# Autodesk Inventor assembly: ASY MSC 080 gills
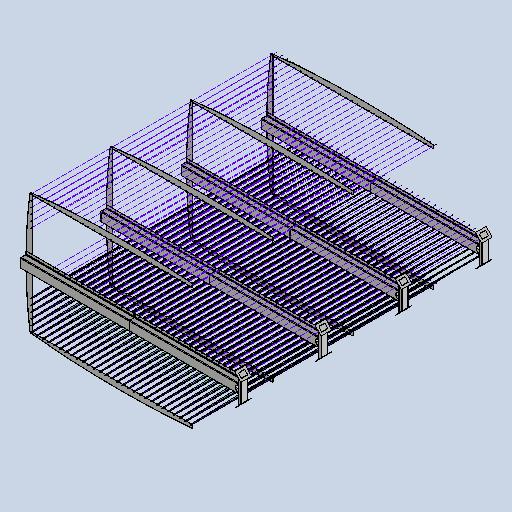
[picture p0: Inventor's stored thumbnail of the model, 512x512]
Saved by Autodesk Inventor 2025 (Build 290162010, 162A)
## iProperties
Created: 2024-08-31
Part Number: ASY MSC 080 gills
Document SubType Name: Assembly
Designer: pokla
Stock Number: ASY МОО 080 Жабры
Author: pokla
## Documents named in this file (20)
- C:\Users\pokla\Documents\Inventor\Отстойник осветлитель\Manturovo_Se-clar-Gleb\ASY MSC Жабры.iam
- C:\Users\pokla\Documents\Inventor\Отстойник осветлитель\Manturovo_Se-clar-Gleb\MSC 802 sheet gills.ipt
- C:\Users\pokla\Documents\Inventor\Отстойник осветлитель\Manturovo_Se-clar-Gleb\MSC 081 pillar gills.ipt
- C:\Users\pokla\Documents\Inventor\Отстойник осветлитель\Manturovo_Se-clar-Gleb\MSC 804 sheet gills.ipt
- C:\Users\pokla\Documents\Inventor\Отстойник осветлитель\Manturovo_Se-clar-Gleb\MSC 803 sheet gills.ipt
- C:\Users\pokla\Documents\Inventor\Отстойник осветлитель\Manturovo_Se-clar-Gleb\MSC 806 sheet gills.ipt
- C:\Users\pokla\Documents\Inventor\Отстойник осветлитель\Manturovo_Se-clar-Gleb\MSC 805 sheet gills.ipt
- C:\Users\pokla\Documents\Inventor\Отстойник осветлитель\Manturovo_Se-clar-Gleb\MSC 808 sheet gills.ipt
- C:\Users\pokla\Documents\Inventor\Отстойник осветлитель\Manturovo_Se-clar-Gleb\MSC 807 sheet gills.ipt
- C:\Users\pokla\Documents\Inventor\Отстойник осветлитель\Manturovo_Se-clar-Gleb\MSC 810 sheet gills.ipt
- C:\Users\pokla\Documents\Inventor\Отстойник осветлитель\Manturovo_Se-clar-Gleb\MSC 809 sheet gills.ipt
- C:\Users\pokla\Documents\Inventor\Отстойник осветлитель\Manturovo_Se-clar-Gleb\MSC 812 sheet gills.ipt
- C:\Users\pokla\Documents\Inventor\Отстойник осветлитель\Manturovo_Se-clar-Gleb\MSC 811 sheet gills.ipt
- C:\Users\pokla\Documents\Inventor\Отстойник осветлитель\Manturovo_Se-clar-Gleb\MSC 084 wall support gills.ipt
- C:\Users\pokla\Documents\Inventor\Отстойник осветлитель\Manturovo_Se-clar-Gleb\MSC 085 bottom support gills.ipt
- C:\Users\pokla\Documents\Inventor\Отстойник осветлитель\Manturovo_Se-clar-Gleb\MSC 082 pillar gills.ipt
- C:\Users\pokla\Documents\Inventor\Отстойник осветлитель\Manturovo_Se-clar-Gleb\MSC 086 string for sheets gills.ipt
- C:\Users\pokla\Documents\Inventor\Отстойник осветлитель\Manturovo_Se-clar-Gleb\MSC 083 top support gills.ipt
- C:\Users\pokla\Documents\Inventor\Отстойник осветлитель\Manturovo_Se-clar-Gleb\MSC 087 bottom plate gills.ipt
- C:\Users\pokla\Documents\Inventor\Отстойник осветлитель\Manturovo_Se-clar-Gleb\MSC 801 sheet gills.ipt
## Components (240 placed, 19 different names)
1. MSC 804 sheet gills:1 — Rigid:39
2. MSC 803 sheet gills:1 — Angle:2, Tangent:8, Tangent:9, Flush:15, Flush:19, Rigid:39
3. MSC 806 sheet gills:1 — Rigid:36
4. MSC 805 sheet gills:1 — Rigid:36, Angle:3, Tangent:10, Tangent:11, Flush:15, Flush:16
5. MSC 808 sheet gills:1 — Rigid:37
6. MSC 807 sheet gills:1 — Rigid:37, Angle:4, Tangent:12, Tangent:13, Flush:16, Flush:17
7. MSC 810 sheet gills:1 — Rigid:38
8. MSC 809 sheet gills:1 — Rigid:38, Angle:5, Tangent:17, Tangent:18, Flush:17, Flush:18
9. MSC 812 sheet gills:1 — Rigid:32
10. MSC 811 sheet gills:1 — Rigid:32, Angle:6, Tangent:19, Tangent:20, Flush:18
11. MSC 084 wall support gills:1 — Rigid:12, Rigid:25, Rigid:30, Tangent:14, Tangent:15
12. MSC 084 wall support gills:2 — Rigid:25, Rigid:26, Mate:17
13. MSC 084 wall support gills:3 — Rigid:26, Rigid:27
14. MSC 084 wall support gills:4 — Rigid:27
15. MSC 085 bottom support gills:1 — Rigid:6, Rigid:7, Flush:12, Mate:12, Flush:14, Mate:15, Mate:16, Flush:9
16. MSC 081 pillar gills:1 — Flush:12, Mate:12, Flush:14, Rotational:1, Rotational:2, Tangent:16
17. MSC 082 pillar gills:1 — Rigid:28, Rigid:29
18. MSC 085 bottom support gills:2
19. MSC 081 pillar gills:2
20. MSC 082 pillar gills:2
21. MSC 085 bottom support gills:3
22. MSC 081 pillar gills:3
23. MSC 082 pillar gills:3
24. MSC 085 bottom support gills:4
25. MSC 081 pillar gills:4
26. MSC 082 pillar gills:4
27. MSC 801 sheet gills:1 — Mate:17, Rigid:33, Angle:2, Angle:3, Angle:4, Angle:5, Angle:6, Tangent:14, Tangent:15, Tangent:16, Flush:19
28. MSC 801 sheet gills:2
29. MSC 801 sheet gills:3
30. MSC 801 sheet gills:4
31. MSC 801 sheet gills:5
32. MSC 801 sheet gills:6
33. MSC 801 sheet gills:7
34. MSC 801 sheet gills:8
35. MSC 801 sheet gills:9
36. MSC 801 sheet gills:10
37. MSC 801 sheet gills:11
38. MSC 801 sheet gills:12
39. MSC 801 sheet gills:13
40. MSC 801 sheet gills:14
41. MSC 801 sheet gills:15
42. MSC 801 sheet gills:16
43. MSC 801 sheet gills:17
44. MSC 801 sheet gills:18
45. MSC 801 sheet gills:19
46. MSC 801 sheet gills:20
47. MSC 801 sheet gills:21
48. MSC 801 sheet gills:22
49. MSC 801 sheet gills:23
50. MSC 801 sheet gills:24
51. MSC 801 sheet gills:25
52. MSC 801 sheet gills:26
53. MSC 801 sheet gills:27
54. MSC 801 sheet gills:28
55. MSC 801 sheet gills:29
56. MSC 802 sheet gills:1 — Rigid:33
57. MSC 802 sheet gills:2
58. MSC 802 sheet gills:3
59. MSC 802 sheet gills:4
60. MSC 802 sheet gills:5
61. MSC 802 sheet gills:6
62. MSC 802 sheet gills:7
63. MSC 802 sheet gills:8
64. MSC 802 sheet gills:9
65. MSC 802 sheet gills:10
66. MSC 802 sheet gills:11
67. MSC 802 sheet gills:12
68. MSC 802 sheet gills:13
69. MSC 802 sheet gills:14
70. MSC 802 sheet gills:15
71. MSC 802 sheet gills:16
72. MSC 802 sheet gills:17
73. MSC 802 sheet gills:18
74. MSC 802 sheet gills:19
75. MSC 802 sheet gills:20
76. MSC 802 sheet gills:21
77. MSC 802 sheet gills:22
78. MSC 802 sheet gills:23
79. MSC 802 sheet gills:24
80. MSC 802 sheet gills:25
81. MSC 802 sheet gills:26
82. MSC 802 sheet gills:27
83. MSC 802 sheet gills:28
84. MSC 802 sheet gills:29
85. MSC 084 wall support gills:5 — Rigid:15, Rigid:31
86. MSC 083 top support gills:1 — Rigid:24, Rigid:29, Rigid:31
87. MSC 083 top support gills:2 — Rigid:28, Rigid:30, Tangent:8, Tangent:9, Tangent:10, Tangent:11, Tangent:12, Tangent:13, Tangent:17, Tangent:18, Tangent:19, Tangent:20, Rigid:40
88. MSC 087 bottom plate gills:1 — Rigid:6
89. MSC 087 bottom plate gills:2 — Rigid:7
90. MSC 084 wall support gills:6
91. MSC 083 top support gills:3
92. MSC 083 top support gills:4
93. MSC 087 bottom plate gills:3
94. MSC 087 bottom plate gills:4
95. MSC 084 wall support gills:7
96. MSC 083 top support gills:5
97. MSC 083 top support gills:6
98. MSC 087 bottom plate gills:5
99. MSC 087 bottom plate gills:6
100. MSC 084 wall support gills:8
101. MSC 083 top support gills:7
102. MSC 083 top support gills:8
103. MSC 087 bottom plate gills:7
104. MSC 087 bottom plate gills:8
105. MSC 086 string for sheets gills:1 — Rigid:12
106. MSC 086 string for sheets gills:2 — Rigid:15
107. MSC 086 string for sheets gills:3
108. MSC 086 string for sheets gills:4
109. MSC 086 string for sheets gills:5
110. MSC 086 string for sheets gills:6
111. MSC 086 string for sheets gills:7
112. MSC 086 string for sheets gills:8
113. MSC 086 string for sheets gills:9
114. MSC 086 string for sheets gills:10
115. MSC 086 string for sheets gills:11
116. MSC 086 string for sheets gills:12
117. MSC 086 string for sheets gills:13
118. MSC 086 string for sheets gills:14
119. MSC 086 string for sheets gills:15
120. MSC 086 string for sheets gills:16
121. MSC 086 string for sheets gills:17
122. MSC 086 string for sheets gills:18
123. MSC 086 string for sheets gills:19
124. MSC 086 string for sheets gills:20
125. MSC 086 string for sheets gills:21
126. MSC 086 string for sheets gills:22
127. MSC 086 string for sheets gills:23
128. MSC 086 string for sheets gills:24
129. MSC 086 string for sheets gills:25
130. MSC 086 string for sheets gills:26
131. MSC 086 string for sheets gills:27
132. MSC 086 string for sheets gills:28
133. MSC 086 string for sheets gills:29
134. MSC 086 string for sheets gills:30
135. MSC 086 string for sheets gills:31
136. MSC 086 string for sheets gills:32
137. MSC 086 string for sheets gills:33
138. MSC 086 string for sheets gills:34
139. MSC 086 string for sheets gills:35
140. MSC 086 string for sheets gills:36
141. MSC 086 string for sheets gills:37
142. MSC 086 string for sheets gills:38
143. MSC 086 string for sheets gills:39
144. MSC 086 string for sheets gills:40
145. MSC 086 string for sheets gills:41
146. MSC 086 string for sheets gills:42
147. MSC 086 string for sheets gills:43
148. MSC 086 string for sheets gills:44
149. MSC 086 string for sheets gills:45
150. MSC 086 string for sheets gills:46
151. MSC 086 string for sheets gills:47
152. MSC 086 string for sheets gills:48
153. MSC 086 string for sheets gills:49
154. MSC 086 string for sheets gills:50
155. MSC 086 string for sheets gills:51
156. MSC 086 string for sheets gills:52
157. MSC 086 string for sheets gills:53
158. MSC 086 string for sheets gills:54
159. MSC 086 string for sheets gills:55
160. MSC 086 string for sheets gills:56
161. MSC 086 string for sheets gills:57 — Rotational:2
162. MSC 086 string for sheets gills:58 — Rotational:1
163. MSC 086 string for sheets gills:59
164. MSC 086 string for sheets gills:60
165. MSC 086 string for sheets gills:61
166. MSC 086 string for sheets gills:62
167. MSC 086 string for sheets gills:63
168. MSC 086 string for sheets gills:64
169. MSC 086 string for sheets gills:65
170. MSC 086 string for sheets gills:66
171. MSC 086 string for sheets gills:67
172. MSC 086 string for sheets gills:68
173. MSC 086 string for sheets gills:69
174. MSC 086 string for sheets gills:70
175. MSC 086 string for sheets gills:71
176. MSC 086 string for sheets gills:72
177. MSC 086 string for sheets gills:73
178. MSC 086 string for sheets gills:74
179. MSC 086 string for sheets gills:75
180. MSC 086 string for sheets gills:76
181. MSC 086 string for sheets gills:77
182. MSC 086 string for sheets gills:78
183. MSC 086 string for sheets gills:79
184. MSC 086 string for sheets gills:80
185. MSC 086 string for sheets gills:81
186. MSC 086 string for sheets gills:82
187. MSC 086 string for sheets gills:83
188. MSC 086 string for sheets gills:84
189. MSC 086 string for sheets gills:85
190. MSC 086 string for sheets gills:86
191. MSC 086 string for sheets gills:87
192. MSC 086 string for sheets gills:88
193. MSC 086 string for sheets gills:89
194. MSC 086 string for sheets gills:90
195. MSC 086 string for sheets gills:91
196. MSC 086 string for sheets gills:92
197. MSC 086 string for sheets gills:93
198. MSC 086 string for sheets gills:94
199. MSC 086 string for sheets gills:95
200. MSC 086 string for sheets gills:96
201. MSC 086 string for sheets gills:97
202. MSC 086 string for sheets gills:98
203. MSC 086 string for sheets gills:99
204. MSC 086 string for sheets gills:100
205. MSC 086 string for sheets gills:101
206. MSC 086 string for sheets gills:102
207. MSC 086 string for sheets gills:103
208. MSC 086 string for sheets gills:104
209. MSC 086 string for sheets gills:105
210. MSC 086 string for sheets gills:106
211. MSC 086 string for sheets gills:107
212. MSC 086 string for sheets gills:108
213. MSC 086 string for sheets gills:109
214. MSC 086 string for sheets gills:110
215. MSC 086 string for sheets gills:111
216. MSC 086 string for sheets gills:112
217. MSC 086 string for sheets gills:113
218. MSC 086 string for sheets gills:114
219. MSC 086 string for sheets gills:115
220. MSC 086 string for sheets gills:116
221. MSC 086 string for sheets gills:117
222. MSC 086 string for sheets gills:118
223. MSC 086 string for sheets gills:119
224. MSC 086 string for sheets gills:120
225. MSC 086 string for sheets gills:121
226. MSC 086 string for sheets gills:122
227. MSC 086 string for sheets gills:123
228. MSC 086 string for sheets gills:124
229. MSC 086 string for sheets gills:125 — Rigid:40
230. MSC 086 string for sheets gills:126
231. MSC 086 string for sheets gills:127
232. MSC 086 string for sheets gills:128
233. MSC 086 string for sheets gills:129
234. MSC 086 string for sheets gills:130
235. MSC 086 string for sheets gills:131 — Rigid:24
236. MSC 086 string for sheets gills:132
237. MSC 086 string for sheets gills:133
238. MSC 086 string for sheets gills:134
239. MSC 086 string for sheets gills:135
240. MSC 086 string for sheets gills:136
## Component patterns: (4 elements, first: MSC 085 bottom support gills:1 + MSC 081 pillar gills:1 + MSC 082 pillar gills:1), (29 elements, first: MSC 801 sheet gills:1), (29 elements, first: MSC 802 sheet gills:1), (4 elements, first: MSC 084 wall support gills:5 + MSC 083 top support gills:1 + MSC 083 top support gills:2 + MSC 087 bottom plate gills:1 + MSC 087 bottom plate gills:2), (28 elements, first: MSC 086 string for sheets gills:1 + MSC 086 string for sheets gills:2), (34 elements, first: MSC 086 string for sheets gills:57 + MSC 086 string for sheets gills:58), (6 elements, first: MSC 086 string for sheets gills:125), (6 elements, first: MSC 086 string for sheets gills:131)
## Relationships (52: WeldJoint 20, Tangent 13, Flush 8, Angle 5, Mate 4, RevoluteJoint 2)
- [WeldJoint]: MSC 081 pillar gills:1 ↔ MSC 082 pillar gills:1
- Rigid:6 [WeldJoint]: MSC 085 bottom support gills:1 ↔ MSC 087 bottom plate gills:1
- Rigid:7 [WeldJoint]: MSC 085 bottom support gills:1 ↔ MSC 087 bottom plate gills:2
- Flush:12: MSC 085 bottom support gills:1 ↔ MSC 081 pillar gills:1
- Mate:12: MSC 085 bottom support gills:1 ↔ MSC 081 pillar gills:1
- Flush:14 (5 mm): MSC 085 bottom support gills:1 ↔ MSC 081 pillar gills:1
- Rigid:12 [WeldJoint] (-5 mm): MSC 084 wall support gills:1 ↔ MSC 086 string for sheets gills:1
- Rigid:15 [WeldJoint] (-5 mm): MSC 084 wall support gills:5 ↔ MSC 086 string for sheets gills:2
- Mate:15: MSC 085 bottom support gills:1
- Mate:16: MSC 085 bottom support gills:1
- Flush:9: MSC 085 bottom support gills:1
- Rigid:24 [WeldJoint] (-5 mm): MSC 083 top support gills:1 ↔ MSC 086 string for sheets gills:131
- Rigid:25 [WeldJoint] (985 mm): MSC 084 wall support gills:1 ↔ MSC 084 wall support gills:2
- Rigid:26 [WeldJoint] (985 mm): MSC 084 wall support gills:2 ↔ MSC 084 wall support gills:3
- Rigid:27 [WeldJoint] (985 mm): MSC 084 wall support gills:3 ↔ MSC 084 wall support gills:4
- Mate:17: MSC 084 wall support gills:2 ↔ MSC 801 sheet gills:1
- Rigid:28 [WeldJoint]: MSC 082 pillar gills:1 ↔ MSC 083 top support gills:2
- Rigid:29 [WeldJoint]: MSC 082 pillar gills:1 ↔ MSC 083 top support gills:1
- Rigid:30 [WeldJoint]: MSC 084 wall support gills:1 ↔ MSC 083 top support gills:2
- Rigid:31 [WeldJoint]: MSC 084 wall support gills:5 ↔ MSC 083 top support gills:1
- Rotational:1 [RevoluteJoint] (5 mm): MSC 081 pillar gills:1 ↔ MSC 086 string for sheets gills:58
- Rotational:2 [RevoluteJoint] (-5 mm): MSC 081 pillar gills:1 ↔ MSC 086 string for sheets gills:57
- Rigid:32 [WeldJoint] (-10 mm): MSC 812 sheet gills:1 ↔ MSC 811 sheet gills:1
- Rigid:33 [WeldJoint] (-10 mm): MSC 801 sheet gills:1 ↔ MSC 802 sheet gills:1
- Rigid:36 [WeldJoint] (-10 mm): MSC 806 sheet gills:1 ↔ MSC 805 sheet gills:1
- Rigid:37 [WeldJoint] (-10 mm): MSC 808 sheet gills:1 ↔ MSC 807 sheet gills:1
- Rigid:38 [WeldJoint] (-10 mm): MSC 810 sheet gills:1 ↔ MSC 809 sheet gills:1
- Angle:2 (0 deg): MSC 803 sheet gills:1 ↔ MSC 801 sheet gills:1
- Angle:3 (0 deg): MSC 805 sheet gills:1 ↔ MSC 801 sheet gills:1
- Angle:4 (0 deg): MSC 807 sheet gills:1 ↔ MSC 801 sheet gills:1
- Angle:5 (0 deg): MSC 809 sheet gills:1 ↔ MSC 801 sheet gills:1
- Angle:6 (0 deg): MSC 811 sheet gills:1 ↔ MSC 801 sheet gills:1
- Tangent:8: MSC 803 sheet gills:1 ↔ MSC 083 top support gills:2
- Tangent:9: MSC 803 sheet gills:1 ↔ MSC 083 top support gills:2
- Tangent:10: MSC 805 sheet gills:1 ↔ MSC 083 top support gills:2
- Tangent:11: MSC 805 sheet gills:1 ↔ MSC 083 top support gills:2
- Tangent:12: MSC 807 sheet gills:1 ↔ MSC 083 top support gills:2
- Tangent:13: MSC 807 sheet gills:1 ↔ MSC 083 top support gills:2
- Tangent:14: MSC 084 wall support gills:1 ↔ MSC 801 sheet gills:1
- Tangent:15: MSC 084 wall support gills:1 ↔ MSC 801 sheet gills:1
- Tangent:16: MSC 081 pillar gills:1 ↔ MSC 801 sheet gills:1
- Tangent:17: MSC 809 sheet gills:1 ↔ MSC 083 top support gills:2
- Tangent:18: MSC 809 sheet gills:1 ↔ MSC 083 top support gills:2
- Tangent:19: MSC 811 sheet gills:1 ↔ MSC 083 top support gills:2
- Tangent:20: MSC 811 sheet gills:1 ↔ MSC 083 top support gills:2
- Flush:15: MSC 803 sheet gills:1 ↔ MSC 805 sheet gills:1
- Flush:16: MSC 805 sheet gills:1 ↔ MSC 807 sheet gills:1
- Flush:17: MSC 807 sheet gills:1 ↔ MSC 809 sheet gills:1
- Flush:18: MSC 809 sheet gills:1 ↔ MSC 811 sheet gills:1
- Flush:19: MSC 803 sheet gills:1 ↔ MSC 801 sheet gills:1
- Rigid:39 [WeldJoint] (-10 mm): MSC 804 sheet gills:1 ↔ MSC 803 sheet gills:1
- Rigid:40 [WeldJoint] (5 mm): MSC 083 top support gills:2 ↔ MSC 086 string for sheets gills:125
